# Autodesk Inventor assembly: recessedCoverslipAssembly_v1
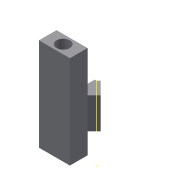
[picture p0: Inventor's stored thumbnail of the model, 180x180]
Saved by Autodesk Inventor 2013 (Build 170138000, 138)
## iProperties
Created: 2014-12-18
Part Number: recessedCoverslipAssembly_v1
Document SubType Name: Assembly
Designer: 120pa
Author: 120pa
## Documents named in this file (3)
- C:\Users\120pa\Desktop\KDean\Coverslip\recessedCoverslipAssembly_v1.iam
- C:\Users\120pa\Desktop\KDean\builtComponents\recessedCoverslip_v1.ipt
- C:\Users\120pa\Desktop\KDean\builtComponents\recessedCoverslipHolder_v1.ipt
## Components (2 placed, 2 different names)
1. recessedCoverslip_v1:1 — Mate:1, Mate:2, Flush:1
2. recessedCoverslipHolder_v1:1 — Mate:1, Mate:2, Flush:1
## Relationships (3: Mate 2, Flush 1)
- Mate:1: recessedCoverslip_v1:1 ↔ recessedCoverslipHolder_v1:1
- Mate:2: recessedCoverslip_v1:1 ↔ recessedCoverslipHolder_v1:1
- Flush:1: recessedCoverslip_v1:1 ↔ recessedCoverslipHolder_v1:1
